# Autodesk Inventor assembly: Assembly
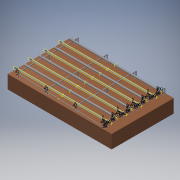
[picture p0: Inventor's stored thumbnail of the model, 180x180]
Saved by Autodesk Inventor 2017 (Build 210142000, 142)
## iProperties
Created: 2017-10-30
Part Number: Assembly
Document SubType Name: Assembly
Designer: DesignPC02
Author: DesignPC02
## Documents named in this file (15)
- C:\Users\DesignPC02\Desktop\hydroponic\Assembly.iam
- C:\Users\DesignPC02\Desktop\hydroponic\wall.ipt
- C:\Users\DesignPC02\Desktop\hydroponic\PipeA.ipt
- C:\Users\DesignPC02\Desktop\hydroponic\Stand.ipt
- C:\Users\DesignPC02\Desktop\hydroponic\PipeB.ipt
- C:\Users\DesignPC02\Desktop\hydroponic\Cap(right).ipt
- C:\Users\DesignPC02\Desktop\hydroponic\water setter.ipt
- C:\Users\DesignPC02\Desktop\hydroponic\90º Elbow.ipt
- C:\Users\DesignPC02\Desktop\hydroponic\Elbow and Tee conector.ipt
- C:\Users\DesignPC02\Desktop\hydroponic\Tee.ipt
- C:\Users\DesignPC02\Desktop\hydroponic\water out put.ipt
- C:\Users\DesignPC02\Desktop\hydroponic\Bottom pipe.ipt
- C:\Users\DesignPC02\Desktop\hydroponic\Cap(left).ipt
- C:\Users\DesignPC02\Desktop\hydroponic\Black part to elbow.ipt
- C:\Users\DesignPC02\Desktop\hydroponic\elbow to tee.ipt
## Components (72 placed, 14 different names)
1. wall:1 — Mate:1, Flush:1, Mate:2, Mate:3, Mate:4, Flush:2, Mate:5, Mate:6, Mate:8, Mate:35
2. Elbow and Tee conector:9 — Mate:36, Mate:37, Mate:38
3. 90º Elbow:9 — Mate:38, Mate:39, Mate:40
4. Bottom pipe:1 — Mate:39, Mate:40
5. elbow to tee:1 — Mate:45
6. Stand:1 — Mate:2, Mate:3, Mate:4, Flush:2, Mate:5, Mate:6, Mate:7, Mate:33, Mate:35
7. Stand:2
8. Stand:3
9. Stand:4 — Mate:14
10. PipeA:1 — Mate:1, Flush:1, Mate:7, Mate:9, Mate:12, Mate:13
11. PipeB:1 — Mate:8, Flush:3, Mate:9
12. PipeA:2
13. PipeB:2
14. PipeA:3
15. PipeB:3
16. PipeA:4
17. PipeB:4
18. Cap(right):1 — Mate:12, Mate:13, Mate:14, Mate:41, Mate:42
19. Cap(right):2
20. Cap(right):3
21. Cap(right):4
22. Cap(right):5
23. Cap(right):6
24. Cap(right):7
25. Cap(right):8
26. Tee:1 — Mate:22, Mate:23, Mate:45
27. Tee:2
28. Tee:3
29. Tee:4
30. Tee:5
31. Tee:6
32. Tee:7
33. Tee:8 — Mate:36, Mate:37
34. water out put:1 — Mate:22, Mate:23
35. water out put:2
36. water out put:3
37. water out put:4
38. water out put:5
39. water out put:6
40. water out put:7
41. Cap(left):1 — Mate:33
42. Cap(left):2
43. Cap(left):3
44. Cap(left):4
45. Cap(left):5
46. Cap(left):6
47. Cap(left):7
48. Cap(left):8
49. water setter:1 — Mate:41, Mate:42, Mate:43
50. water setter:2
51. water setter:3
52. water setter:4
53. water setter:5
54. water setter:6
55. water setter:7
56. water setter:8
57. Black part to elbow:1 — Mate:43, Mate:44
58. Black part to elbow:2
59. Black part to elbow:3
60. Black part to elbow:4
61. Black part to elbow:5
62. Black part to elbow:6
63. Black part to elbow:7
64. Black part to elbow:8
65. 90º Elbow:10 — Mate:44
66. 90º Elbow:11
67. 90º Elbow:12
68. 90º Elbow:13
69. 90º Elbow:14
70. 90º Elbow:15
71. 90º Elbow:16
72. 90º Elbow:17
## Component patterns: (4 elements, first: Stand:1), (4 elements, first: PipeA:1 + PipeB:1), (8 elements, first: Cap(right):1), (8 elements, first: Tee:1), (7 elements, first: water out put:1), (8 elements, first: Cap(left):1), (8 elements, first: water setter:1), (8 elements, first: Black part to elbow:1), (8 elements, first: 90º Elbow:10)
## Relationships (29: Mate 26, Flush 3)
- Mate:1 (267 mm): wall:1 ↔ PipeA:1
- Flush:1: wall:1 ↔ PipeA:1
- Mate:2: wall:1 ↔ Stand:1
- Mate:3: wall:1 ↔ Stand:1
- Mate:4: wall:1 ↔ Stand:1
- Flush:2 (-1964.5 mm): wall:1 ↔ Stand:1
- Mate:5: wall:1 ↔ Stand:1
- Mate:6: wall:1 ↔ Stand:1
- Mate:7: Stand:1 ↔ PipeA:1
- Mate:8 (267 mm): wall:1 ↔ PipeB:1
- Flush:3: PipeB:1
- Mate:9 (338 mm): PipeA:1 ↔ PipeB:1
- Mate:12: PipeA:1 ↔ Cap(right):1
- Mate:13: PipeA:1 ↔ Cap(right):1
- Mate:14 (18 mm): Stand:4 ↔ Cap(right):1
- Mate:22: Tee:1 ↔ water out put:1
- Mate:23 (119 mm): Tee:1 ↔ water out put:1
- Mate:33 (3 mm): Stand:1 ↔ Cap(left):1
- Mate:35: wall:1 ↔ Stand:1
- Mate:36: Elbow and Tee conector:9 ↔ Tee:8
- Mate:37: Elbow and Tee conector:9 ↔ Tee:8
- Mate:38: Elbow and Tee conector:9 ↔ 90º Elbow:9
- Mate:39: 90º Elbow:9 ↔ Bottom pipe:1
- Mate:40 (1975 mm): 90º Elbow:9 ↔ Bottom pipe:1
- Mate:41: Cap(right):1 ↔ water setter:1
- Mate:42 (-38 mm): Cap(right):1 ↔ water setter:1
- Mate:43: water setter:1 ↔ Black part to elbow:1
- Mate:44: Black part to elbow:1 ↔ 90º Elbow:10
- Mate:45: elbow to tee:1 ↔ Tee:1
